# Autodesk Inventor assembly: VexPro Ball Shifter 2 stage 110 mm Shaft
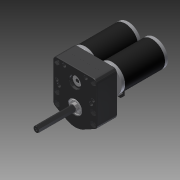
[picture p0: Inventor's stored thumbnail of the model, 180x180]
Saved by Autodesk Inventor 2013 (Build 170138000, 138)
## iProperties
Created: 2013-04-08
Part Number: VexPro Ball Shifter 2 stage 110 mm Shaft
Document SubType Name: Assembly
Designer: Niemitalo_Dan
Author: Niemitalo_Dan
## Documents named in this file (16)
- \\lmss\students\Robotics\CAD Files\COTS Parts\Gearboxes\VexPro Ball Shifter 2 stage 110 mm Shaft.iam
- \\lmss\students\Robotics\CAD Files\COTS Parts\Gearboxes\Components\VexPro Ball Shifters\Ball Shifter Housing - Motor Side.ipt
- \\lmss\students\Robotics\CAD Files\COTS Parts\Bearings - VexPro\Flanged Bearing - 0.75in x 1.375in x .437in.ipt
- \\lmss\students\Robotics\CAD Files\COTS Parts\Bearings - VexPro\Flanged Bearing - 0.5in Round ID x 1.125in OD.ipt
- \\lmss\students\Robotics\CAD Files\COTS Parts\Gearboxes\Components\VexPro Ball Shifters\Ball Shifter Housing - Output Side.ipt
- \\lmss\students\Robotics\CAD Files\COTS Parts\Bearings - VexPro\Flanged Bearing - 0.375in Round ID x 0.875in OD.ipt
- \\lmss\students\Robotics\CAD Files\COTS Parts\Gearboxes\Components\VexPro Ball Shifters\Ballshifter 375 hex cluster shaft.ipt
- \\lmss\students\Robotics\CAD Files\COTS Parts\Gears - VexPro\Gear 20dp 375hex 24T Vex.ipt
- \\lmss\students\Robotics\CAD Files\COTS Parts\Gears - VexPro\Gear 20dp 375hex 40T Vex.ipt
- \\lmss\students\Robotics\CAD Files\COTS Parts\Gearboxes\Components\VexPro Ball Shifters\CIM for Ballshifter.iam
- \\lmss\students\Robotics\CAD Files\COTS Parts\Fasteners\6-32 SHCS x250.ipt
- \\lmss\students\Robotics\CAD Files\COTS Parts\Gearboxes\Components\VexPro Ball Shifters\Shifting Cylinder Mechanism for Ball Shifter.iam
- \\lmss\students\Robotics\CAD Files\COTS Parts\Gearboxes\Components\VexPro Ball Shifters\Ball shifter cluster shaft spacer.ipt
- \\lmss\students\Robotics\CAD Files\COTS Parts\Fasteners\8-32 locknut.ipt
- \\lmss\students\Robotics\CAD Files\COTS Parts\Fasteners\8-32 BHCS x1750.ipt
- \\lmss\students\Robotics\CAD Files\COTS Parts\Gearboxes\Components\VexPro Ball Shifters\Ball Shifter shifting 110mm shaft with gears.iam
## Components (20 placed, 15 different names)
1. Ball Shifter Housing - Motor Side:1 — Insert:1, Mate:1, Mate:2, Insert:4, Insert:9, Mate:3, Insert:10, Mate:4, Mate:5, Mate:6, Mate:7, Mate:8, Insert:14, Insert:15, Mate:10
2. Ball Shifter Housing - Output Side:1 — Mate:1, Mate:2, Insert:3, Insert:5, Mate:5, Insert:12, Insert:13, Mate:10
3. Flanged Bearing - 0.75in x 1.375in x .437in:1 — Insert:3
4. Flanged Bearing - 0.5in Round ID x 1.125in OD:1 — Insert:1, Insert:2
5. Ball Shifter shifting 110mm shaft with gears:1 [sub-assembly] — Insert:2, Mate:9
6. Flanged Bearing - 0.375in Round ID x 0.875in OD:1 — Insert:5
7. Flanged Bearing - 0.375in Round ID x 0.875in OD:2 — Insert:4, Insert:6, Insert:7
8. Ballshifter 375 hex cluster shaft:1 — Insert:6, Angle:1, Angle:2
9. Gear 20dp 375hex 24T Vex:1 — Insert:8, Angle:2, Insert:11
10. Gear 20dp 375hex 40T Vex:1 — Insert:7, Angle:1, Insert:8
11. CIM for Ballshifter:1 [sub-assembly] — Insert:10, Mate:4
12. CIM for Ballshifter:2 [sub-assembly] — Insert:9, Mate:3
13. 6-32 SHCS x250:1
14. 6-32 SHCS x250:2
15. Shifting Cylinder Mechanism for Ball Shifter:1 [sub-assembly] — Mate:6, Mate:7, Mate:8, Mate:9
16. Ball shifter cluster shaft spacer:1 — Insert:11
17. 8-32 locknut:1 — Insert:14
18. 8-32 locknut:2 — Insert:15
19. 8-32 BHCS x1750:1 — Insert:13
20. 8-32 BHCS x1750:2 — Insert:12
## Relationships (27: Insert 15, Mate 10, Angle 2)
- Insert:1: Ball Shifter Housing - Motor Side:1 ↔ Flanged Bearing - 0.5in Round ID x 1.125in OD:1
- Insert:2: Flanged Bearing - 0.5in Round ID x 1.125in OD:1 ↔ Ball Shifter shifting 110mm shaft with gears:1
- Mate:1: Ball Shifter Housing - Motor Side:1 ↔ Ball Shifter Housing - Output Side:1
- Mate:2: Ball Shifter Housing - Motor Side:1 ↔ Ball Shifter Housing - Output Side:1
- Insert:3: Ball Shifter Housing - Output Side:1 ↔ Flanged Bearing - 0.75in x 1.375in x .437in:1
- Insert:4: Ball Shifter Housing - Motor Side:1 ↔ Flanged Bearing - 0.375in Round ID x 0.875in OD:2
- Insert:5: Ball Shifter Housing - Output Side:1 ↔ Flanged Bearing - 0.375in Round ID x 0.875in OD:1
- Insert:6: Flanged Bearing - 0.375in Round ID x 0.875in OD:2 ↔ Ballshifter 375 hex cluster shaft:1
- Insert:7: Flanged Bearing - 0.375in Round ID x 0.875in OD:2 ↔ Gear 20dp 375hex 40T Vex:1
- Angle:1 (0 deg): Ballshifter 375 hex cluster shaft:1 ↔ Gear 20dp 375hex 40T Vex:1
- Insert:8 (1.5875 mm): Gear 20dp 375hex 24T Vex:1 ↔ Gear 20dp 375hex 40T Vex:1
- Angle:2 (0 deg): Ballshifter 375 hex cluster shaft:1 ↔ Gear 20dp 375hex 24T Vex:1
- Insert:9: Ball Shifter Housing - Motor Side:1 ↔ CIM for Ballshifter:2
- Mate:3: Ball Shifter Housing - Motor Side:1 ↔ CIM for Ballshifter:2
- Insert:10: Ball Shifter Housing - Motor Side:1 ↔ CIM for Ballshifter:1
- Mate:4: Ball Shifter Housing - Motor Side:1 ↔ CIM for Ballshifter:1
- Mate:5: Ball Shifter Housing - Motor Side:1 ↔ Ball Shifter Housing - Output Side:1
- Mate:6: Ball Shifter Housing - Motor Side:1 ↔ Shifting Cylinder Mechanism for Ball Shifter:1
- Mate:7: Ball Shifter Housing - Motor Side:1 ↔ Shifting Cylinder Mechanism for Ball Shifter:1
- Mate:8: Ball Shifter Housing - Motor Side:1 ↔ Shifting Cylinder Mechanism for Ball Shifter:1
- Mate:9: Ball Shifter shifting 110mm shaft with gears:1 ↔ Shifting Cylinder Mechanism for Ball Shifter:1
- Insert:11: Gear 20dp 375hex 24T Vex:1 ↔ Ball shifter cluster shaft spacer:1
- Insert:12: Ball Shifter Housing - Output Side:1 ↔ 8-32 BHCS x1750:2
- Insert:13: Ball Shifter Housing - Output Side:1 ↔ 8-32 BHCS x1750:1
- Insert:14: Ball Shifter Housing - Motor Side:1 ↔ 8-32 locknut:1
- Insert:15: Ball Shifter Housing - Motor Side:1 ↔ 8-32 locknut:2
- Mate:10: Ball Shifter Housing - Motor Side:1 ↔ Ball Shifter Housing - Output Side:1
